# Autodesk Inventor assembly: Electric-Scooter
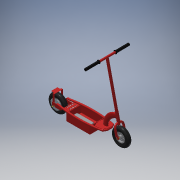
[picture p0: Inventor's stored thumbnail of the model, 180x180]
Saved by Autodesk Inventor 2018 (Build 220112000, 112)
## iProperties
Created: 2018-08-10
Part Number: Electric-Scooter
Document SubType Name: Assembly
Designer: ruben
Author: ruben
## Documents named in this file (10)
- C:\Users\ruben\Documents\Inventor\Electric-Scooter\Electric-Scooter.iam
- C:\Users\ruben\Documents\Inventor\Electric-Scooter\Frame\Frame.iam
- C:\Users\ruben\Documents\Inventor\Electric-Scooter\Transmission\Rear Wheel Axle.ipt
- C:\Users\ruben\Documents\Inventor\Electric-Scooter\Transmission\Real Wheel + Sprocket.iam
- C:\Users\ruben\Documents\Inventor\Electric-Scooter\Transmission\Motor + sprocket + translock.iam
- C:\Users\ruben\Documents\Inventor\Electric-Scooter\Transmission\Motor holder.ipt
- C:\Users\ruben\Documents\Inventor\Electric-Scooter\Frame\Batterybox 2\Waterproof box 2.ipt
- C:\Users\ruben\Documents\Inventor\Electric-Scooter\Wheels\Wheel.iam
- C:\Users\ruben\Documents\Inventor\Electric-Scooter\Transmission\Front Wheel Axle.ipt
- C:\Users\ruben\Documents\Inventor\Electric-Scooter\Frame\Handle bars\Handle bars handles.ipt
## Components (10 placed, 9 different names)
1. Frame:1 [sub-assembly] — Insert:1, Mate:6, Mate:7, Mate:8, Flush:2, Insert:5, Insert:7, Insert:8
2. Real Wheel + Sprocket:1 [sub-assembly] — Insert:2, Flush:1
3. Motor + sprocket + translock:1 [sub-assembly] — Flush:1, Insert:3, Insert:4
4. Motor holder:1 — Insert:3, Insert:4, Flush:2
5. Waterproof box 2:1 — Mate:6, Mate:7, Mate:8
6. Wheel:1 [sub-assembly] — Insert:6
7. Front Wheel Axle:1 — Insert:5, Insert:6
8. Rear Wheel Axle:1 — Insert:1, Insert:2
9. Handle bars handles:1 — Insert:8
10. Handle bars handles:2 — Insert:7
## Relationships (13: Insert 8, Mate 3, Flush 2)
- Insert:1 (0.5 mm): Frame:1 ↔ Rear Wheel Axle:1
- Insert:2 (8.4 mm): Real Wheel + Sprocket:1 ↔ Rear Wheel Axle:1
- Flush:1: Real Wheel + Sprocket:1 ↔ Motor + sprocket + translock:1
- Insert:3: Motor + sprocket + translock:1 ↔ Motor holder:1
- Insert:4: Motor + sprocket + translock:1 ↔ Motor holder:1
- Mate:6 (1 mm): Frame:1 ↔ Waterproof box 2:1
- Mate:7 (32.5 mm): Frame:1 ↔ Waterproof box 2:1
- Mate:8: Frame:1 ↔ Waterproof box 2:1
- Flush:2: Frame:1 ↔ Motor holder:1
- Insert:5 (0.5 mm): Frame:1 ↔ Front Wheel Axle:1
- Insert:6 (6.5 mm): Wheel:1 ↔ Front Wheel Axle:1
- Insert:7: Frame:1 ↔ Handle bars handles:2
- Insert:8: Frame:1 ↔ Handle bars handles:1
